# Autodesk Inventor assembly: servo
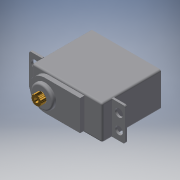
[picture p0: Inventor's stored thumbnail of the model, 180x180]
Saved by Autodesk Inventor 2018 (Build 220112000, 112)
## iProperties
Created: 2017-10-08
Part Number: servo
Document SubType Name: Assembly
Designer: liamg
Author: liamg
## Documents named in this file (3)
- C:\Users\liamg\Desktop\Rotor\Servo moteur\servo.iam
- C:\Users\liamg\Desktop\Rotor\Servo moteur\Corps.ipt
- C:\Users\liamg\Desktop\Rotor\Servo moteur\servo_spine.ipt
## Components (2 placed, 2 different names)
1. Corps:1 — Rotational:1
2. servo_spine:1 — Rotational:1
## Relationships (1: RevoluteJoint 1)
- Rotational:1 [RevoluteJoint]: Corps:1 ↔ servo_spine:1
